# Autodesk Inventor assembly: exhaust header left
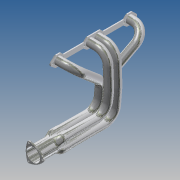
[picture p0: Inventor's stored thumbnail of the model, 180x180]
Saved by Autodesk Inventor 2013 (Build 170138000, 138)
## iProperties
Created: 2013-02-09
Part Number: exhaust header left
Document SubType Name: Assembly
Designer: zhaphod
Author: zhaphod
## Documents named in this file (7)
- C:\drawings\vette\chevy engine\exhaust header left.iam
- C:\drawings\vette\chevy engine\exhaust header plate.ipt
- C:\drawings\vette\chevy engine\exhaust header right pipe 8.ipt
- C:\drawings\vette\chevy engine\exhaust header right pipe 6.ipt
- C:\drawings\vette\chevy engine\exhaust header right pipe 4.ipt
- C:\drawings\vette\chevy engine\exhaust header right pipe 2.ipt
- C:\drawings\vette\chevy engine\exhaust header collector.ipt
## Components (6 placed, 6 different names)
1. exhaust header plate:1 — Mate:1, Flush:1, Mate:2, Mate:3, Mate:4, Flush:2, Flush:3, Flush:4
2. exhaust header right pipe 8:1 — Mate:1, Flush:1, Mate:5, Mate:7
3. exhaust header right pipe 6:1 — Mate:3, Flush:4
4. exhaust header right pipe 4:1 — Mate:2, Flush:3
5. exhaust header right pipe 2:1 — Mate:4, Flush:2, Mate:8
6. exhaust header collector:1 — Mate:5, Mate:7, Mate:8
## Relationships (11: Mate 7, Flush 4)
- Mate:1: exhaust header plate:1 ↔ exhaust header right pipe 8:1
- Flush:1: exhaust header plate:1 ↔ exhaust header right pipe 8:1
- Mate:2: exhaust header plate:1 ↔ exhaust header right pipe 4:1
- Mate:3: exhaust header plate:1 ↔ exhaust header right pipe 6:1
- Mate:4: exhaust header plate:1 ↔ exhaust header right pipe 2:1
- Flush:2: exhaust header plate:1 ↔ exhaust header right pipe 2:1
- Flush:3: exhaust header plate:1 ↔ exhaust header right pipe 4:1
- Flush:4: exhaust header plate:1 ↔ exhaust header right pipe 6:1
- Mate:5: exhaust header right pipe 8:1 ↔ exhaust header collector:1
- Mate:7 (-38.1 mm): exhaust header right pipe 8:1 ↔ exhaust header collector:1
- Mate:8: exhaust header right pipe 2:1 ↔ exhaust header collector:1
